# Autodesk Inventor assembly: base_wall_added
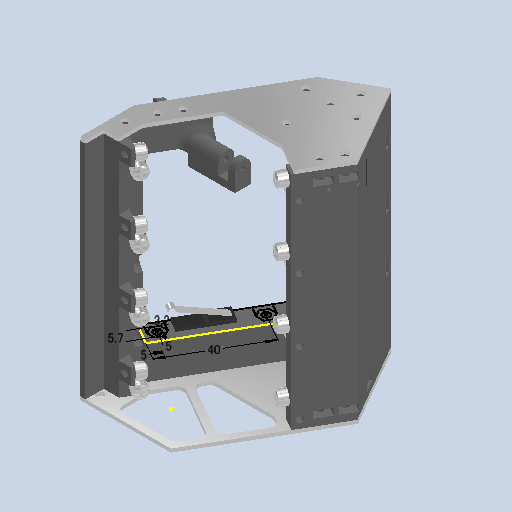
[picture p0: Inventor's stored thumbnail of the model, 512x512]
Saved by Autodesk Inventor 2024.1 (Build 281209000, 209)
## iProperties
Created: 2025-01-18
Part Number: base_wall_added
Document SubType Name: Assembly
Designer: hibik
Author: hibik
## Documents named in this file (3)
- C:\Users\hibik\Documents\Robomech\RESCUE\ORCA\hard\fork\right\base_wall_added.iam
- C:\Users\hibik\Documents\Robomech\RESCUE\ORCA\hard\fork\right\base.iam
- C:\Users\hibik\Documents\Robomech\RESCUE\ORCA\hard\fork\right\base_backwall_setter_upper.ipt
## Components (2 placed, 2 different names)
1. base:1 [sub-assembly] — フラッシュ:1, フラッシュ:2, メイト:1
2. base_backwall_setter_upper:1 — フラッシュ:1, フラッシュ:2, メイト:1
## Relationships (3: Flush 2, Mate 1)
- フラッシュ:1 [Flush]: base:1 ↔ base_backwall_setter_upper:1
- フラッシュ:2 [Flush]: base:1 ↔ base_backwall_setter_upper:1
- メイト:1 [Mate]: base:1 ↔ base_backwall_setter_upper:1
